# Autodesk Inventor assembly: 3_5mm_5_08mm_adapter_assembly
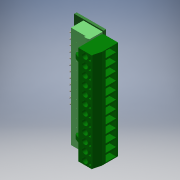
[picture p0: Inventor's stored thumbnail of the model, 180x180]
Saved by Autodesk Inventor 2018 (Build 220112000, 112)
## iProperties
Created: 2018-09-24
Part Number: 3_5mm_5_08mm_adapter_assembly
Document SubType Name: Assembly
Designer: Rich
Author: Rich
## Documents named in this file (5)
- C:\Users\Rich\development\UWaterloo\power-distro.git\SolidModels\3_5mm_5_08mm_adapter_assembly.iam
- C:\Users\Rich\development\UWaterloo\power-distro.git\SolidModels\Phoenix_1945193.ipt
- C:\Users\Rich\development\UWaterloo\power-distro.git\SolidModels\3_5MM_TO_5_08MM_ADAPTOR_PCB.ipt
- C:\Users\Rich\development\UWaterloo\power-distro.git\SolidModels\OST_EDSTLZ950-12.ipt
- C:\Users\Rich\development\UWaterloo\power-distro.git\SolidModels\OST_OSTJ125153.ipt
## Components (4 placed, 4 different names)
1. Phoenix_1945193:1 — Mate:20, Mate:21, Mate:22
2. 3_5MM_TO_5_08MM_ADAPTOR_PCB:1 — Flush:1, Flush:2, Flush:3, Mate:10, Mate:20, Mate:21, Mate:22, Mate:23, Mate:24
3. OST_EDSTLZ950-12:1 — Mate:10, Mate:13, Mate:14, Mate:15, Mate:23, Mate:24
4. OST_OSTJ125153:1 — Mate:13, Mate:14, Mate:15
## Relationships (12: Mate 9, Flush 3)
- Flush:1: 3_5MM_TO_5_08MM_ADAPTOR_PCB:1
- Flush:2: 3_5MM_TO_5_08MM_ADAPTOR_PCB:1
- Flush:3: 3_5MM_TO_5_08MM_ADAPTOR_PCB:1
- Mate:10: 3_5MM_TO_5_08MM_ADAPTOR_PCB:1 ↔ OST_EDSTLZ950-12:1
- Mate:13: OST_EDSTLZ950-12:1 ↔ OST_OSTJ125153:1
- Mate:14: OST_EDSTLZ950-12:1 ↔ OST_OSTJ125153:1
- Mate:15: OST_EDSTLZ950-12:1 ↔ OST_OSTJ125153:1
- Mate:20: Phoenix_1945193:1 ↔ 3_5MM_TO_5_08MM_ADAPTOR_PCB:1
- Mate:21: Phoenix_1945193:1 ↔ 3_5MM_TO_5_08MM_ADAPTOR_PCB:1
- Mate:22: Phoenix_1945193:1 ↔ 3_5MM_TO_5_08MM_ADAPTOR_PCB:1
- Mate:23: 3_5MM_TO_5_08MM_ADAPTOR_PCB:1 ↔ OST_EDSTLZ950-12:1
- Mate:24: 3_5MM_TO_5_08MM_ADAPTOR_PCB:1 ↔ OST_EDSTLZ950-12:1
